# Autodesk Inventor assembly: Ball Screw Nut
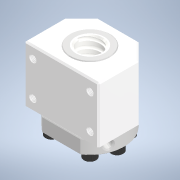
[picture p0: Inventor's stored thumbnail of the model, 180x180]
Saved by Autodesk Inventor 2022.3 (Build 263350000, 350)
## iProperties
Created: 2022-04-29
Part Number: Ball Screw Nut
Document SubType Name: Assembly
Designer: Robert Nies
Sending System: Autodesk Translation Framework v10.14.0.1471
Preprocessor: ST-DEVELOPER v18.1
Title: G:/My Drive/Misc/Misc 3D Files/Mechanical Stuff/SFU1605 Drive Assembly.step
## Documents named in this file (4)
- C:\Users\rober\PycharmProjects\CNCRouter\Stock Parts\Linear Motion\Ball Screw Nut.iam
- C:\Users\rober\PycharmProjects\CNCRouter\Stock Parts\Linear Motion\SFU1605 Ball Screw Nut v2.ipt
- C:\Users\rober\PycharmProjects\CNCRouter\Stock Parts\Linear Motion\DSG16H Ball Nut Housing v3.ipt
- C:\Users\rober\PycharmProjects\CNCRouter\Stock Parts\Linear Motion\M5 x 20 Socket Head Screw.ipt
## Components (8 placed, 3 different names)
1. SFU1605 Ball Screw Nut v2:1 — Rotational:2, Flush:1, Rotational:3, Rotational:4, Rotational:5, Rotational:6, Rotational:7, Rotational:8
2. DSG16H Ball Nut Housing v3:1 — Rotational:2, Flush:1
3. M5 x 20 Socket Head Screw:1 — Rotational:6
4. M5 x 20 Socket Head Screw:2 — Rotational:4
5. M5 x 20 Socket Head Screw:3 — Rotational:3
6. M5 x 20 Socket Head Screw:4 — Rotational:7
7. M5 x 20 Socket Head Screw:5 — Rotational:8
8. M5 x 20 Socket Head Screw:6 — Rotational:5
## Relationships (8: RevoluteJoint 7, Flush 1)
- Rotational:2 [RevoluteJoint]: SFU1605 Ball Screw Nut v2:1 ↔ DSG16H Ball Nut Housing v3:1
- Flush:1: SFU1605 Ball Screw Nut v2:1 ↔ DSG16H Ball Nut Housing v3:1
- Rotational:3 [RevoluteJoint]: SFU1605 Ball Screw Nut v2:1 ↔ M5 x 20 Socket Head Screw:3
- Rotational:4 [RevoluteJoint]: SFU1605 Ball Screw Nut v2:1 ↔ M5 x 20 Socket Head Screw:2
- Rotational:5 [RevoluteJoint]: SFU1605 Ball Screw Nut v2:1 ↔ M5 x 20 Socket Head Screw:6
- Rotational:6 [RevoluteJoint]: SFU1605 Ball Screw Nut v2:1 ↔ M5 x 20 Socket Head Screw:1
- Rotational:7 [RevoluteJoint]: SFU1605 Ball Screw Nut v2:1 ↔ M5 x 20 Socket Head Screw:4
- Rotational:8 [RevoluteJoint]: SFU1605 Ball Screw Nut v2:1 ↔ M5 x 20 Socket Head Screw:5
